# Autodesk Inventor assembly: Walls
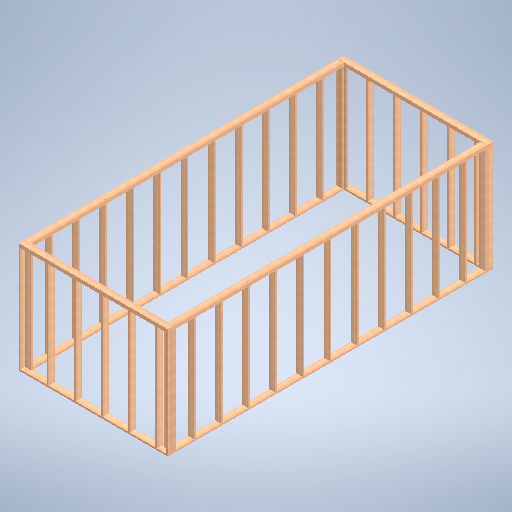
[picture p0: Inventor's stored thumbnail of the model, 512x512]
Saved by Autodesk Inventor 2025 (Build 290162010, 162A)
## iProperties
Created: 2024-09-15
Part Number: Walls
Document SubType Name: Assembly
Designer: Tom
Author: Tom
## Documents named in this file (10)
- C:\Users\Tom\Documents\Inventor\Mobility\Additional_Building\Walls.iam
- C:\Users\Tom\Documents\Inventor\Mobility\Additional_Building\Plate_With_Length_144_Inches.ipt
- C:\Users\Tom\Documents\Inventor\Mobility\Additional_Building\Plate_With_Length_121_Inches.ipt
- C:\Users\Tom\Documents\Inventor\Mobility\Additional_Building\California_Corner.iam
- C:\Users\Tom\Documents\Inventor\Mobility\Additional_Building\California_Corner_MIR.iam
- C:\Users\Tom\Documents\Inventor\Mobility\Additional_Building\California_Corner_MIR1.iam
- C:\Users\Tom\Documents\Inventor\Mobility\Additional_Building\California_Corner_MIR_MIR.iam
- C:\Users\Tom\Documents\Inventor\Mobility\Additional_Building\Stud_With_Height_93_Inches.ipt
- C:\Users\Tom\Documents\Inventor\Mobility\Additional_Building\Plate_With_Length_132_Inches.ipt
- C:\Users\Tom\Documents\Inventor\Mobility\Additional_Building\Plate_With_Length_66.5_Inches.ipt
## Components (56 placed, 9 different names)
1. California_Corner:1 [sub-assembly] — Mate:2, Flush:3, Flush:4
2. California_Corner_MIR:1 [sub-assembly] — Mate:5, Mate:6, Flush:8
3. California_Corner_MIR1:1 [sub-assembly]
4. California_Corner_MIR_MIR:1 [sub-assembly]
5. Plate_With_Length_132_Inches:1 — Mate:8, Flush:9, Flush:10, Mate:10
6. Plate_With_Length_132_Inches:2
7. Plate_With_Length_144_Inches:9 — Mate:11, Mate:12, Flush:12
8. Plate_With_Length_144_Inches:10
9. Plate_With_Length_144_Inches:1 — Flush:5
10. Plate_With_Length_144_Inches:2
11. Plate_With_Length_144_Inches:3 — Mate:1, Flush:1, Flush:2, Mate:4, Flush:6, Flush:8
12. Plate_With_Length_144_Inches:4 — Mate:2, Flush:3, Flush:4
13. Plate_With_Length_121_Inches:1 — Mate:1, Flush:1, Flush:2, Mate:3, Mate:7
14. Plate_With_Length_121_Inches:2
15. Plate_With_Length_144_Inches:5 — Flush:9
16. Plate_With_Length_144_Inches:6
17. Plate_With_Length_144_Inches:7 — Mate:9, Flush:11
18. Plate_With_Length_144_Inches:8 — Mate:11, Flush:12
19. Plate_With_Length_121_Inches:3 — Flush:7, Mate:8, Flush:10
20. Plate_With_Length_121_Inches:4
21. Stud_With_Height_93_Inches:1 — Mate:4, Flush:6, Mate:5
22. Stud_With_Height_93_Inches:2
23. Stud_With_Height_93_Inches:3
24. Stud_With_Height_93_Inches:4
25. Stud_With_Height_93_Inches:5
26. Stud_With_Height_93_Inches:6
27. Stud_With_Height_93_Inches:7
28. Stud_With_Height_93_Inches:8
29. Stud_With_Height_93_Inches:9
30. Stud_With_Height_93_Inches:10
31. Stud_With_Height_93_Inches:11
32. Stud_With_Height_93_Inches:12
33. Stud_With_Height_93_Inches:13
34. Stud_With_Height_93_Inches:14
35. Stud_With_Height_93_Inches:15
36. Stud_With_Height_93_Inches:16
37. Stud_With_Height_93_Inches:17
38. Stud_With_Height_93_Inches:18
39. Stud_With_Height_93_Inches:19
40. Stud_With_Height_93_Inches:20
41. Stud_With_Height_93_Inches:21
42. Stud_With_Height_93_Inches:22
43. Stud_With_Height_93_Inches:23 — Flush:7, Mate:6, Mate:7
44. Stud_With_Height_93_Inches:24
45. Stud_With_Height_93_Inches:25
46. Stud_With_Height_93_Inches:26
47. Stud_With_Height_93_Inches:27
48. Stud_With_Height_93_Inches:28
49. Stud_With_Height_93_Inches:29
50. Stud_With_Height_93_Inches:30
51. Stud_With_Height_93_Inches:31
52. Stud_With_Height_93_Inches:32
53. Plate_With_Length_66.5_Inches:1 — Mate:9, Mate:10, Flush:11
54. Plate_With_Length_66.5_Inches:2 — Mate:12
55. Plate_With_Length_66.5_Inches:3
56. Plate_With_Length_66.5_Inches:4
## Component patterns: (2 elements), (2 elements), (2 elements), (2 elements, first: Plate_With_Length_132_Inches:1), (2 elements, first: Plate_With_Length_144_Inches:9), (4 elements, first: Plate_With_Length_144_Inches:1), (2 elements, first: Plate_With_Length_121_Inches:1), Component Pattern 1:2 (4 elements), Component Pattern 2:2 (2 elements), (11 elements, first: Stud_With_Height_93_Inches:1), Component Pattern 4:2 (11 elements), (5 elements, first: Stud_With_Height_93_Inches:23), Component Pattern 6:2 (5 elements), (2 elements, first: Plate_With_Length_66.5_Inches:1), Component Pattern 10:2 (2 elements)
## Relationships (24: Mate 12, Flush 12)
- Mate:1: Plate_With_Length_144_Inches:3 ↔ Plate_With_Length_121_Inches:1
- Flush:1: Plate_With_Length_144_Inches:3 ↔ Plate_With_Length_121_Inches:1
- Flush:2: Plate_With_Length_144_Inches:3 ↔ Plate_With_Length_121_Inches:1
- Mate:2: California_Corner:1 ↔ Plate_With_Length_144_Inches:4
- Flush:3: California_Corner:1 ↔ Plate_With_Length_144_Inches:4
- Flush:4: California_Corner:1 ↔ Plate_With_Length_144_Inches:4
- Flush:5: Plate_With_Length_144_Inches:1
- Mate:3 (1536.7 mm): Plate_With_Length_121_Inches:1
- Mate:4: Plate_With_Length_144_Inches:3 ↔ Stud_With_Height_93_Inches:1
- Flush:6: Plate_With_Length_144_Inches:3 ↔ Stud_With_Height_93_Inches:1
- Mate:5 (412.75 mm): California_Corner_MIR:1 ↔ Stud_With_Height_93_Inches:1
- Flush:7: Plate_With_Length_121_Inches:3 ↔ Stud_With_Height_93_Inches:23
- Mate:6 (590.55 mm): California_Corner_MIR:1 ↔ Stud_With_Height_93_Inches:23
- Mate:7: Plate_With_Length_121_Inches:1 ↔ Stud_With_Height_93_Inches:23
- Flush:8: California_Corner_MIR:1 ↔ Plate_With_Length_144_Inches:3
- Mate:8: Plate_With_Length_132_Inches:1 ↔ Plate_With_Length_121_Inches:3
- Flush:9: Plate_With_Length_132_Inches:1 ↔ Plate_With_Length_144_Inches:5
- Flush:10: Plate_With_Length_132_Inches:1 ↔ Plate_With_Length_121_Inches:3
- Mate:9: Plate_With_Length_144_Inches:7 ↔ Plate_With_Length_66.5_Inches:1
- Mate:10: Plate_With_Length_132_Inches:1 ↔ Plate_With_Length_66.5_Inches:1
- Flush:11: Plate_With_Length_144_Inches:7 ↔ Plate_With_Length_66.5_Inches:1
- Mate:11: Plate_With_Length_144_Inches:9 ↔ Plate_With_Length_144_Inches:8
- Mate:12: Plate_With_Length_144_Inches:9 ↔ Plate_With_Length_66.5_Inches:2
- Flush:12: Plate_With_Length_144_Inches:9 ↔ Plate_With_Length_144_Inches:8
